# Autodesk Inventor assembly: Toughbox Nanotube 31 full gear drive
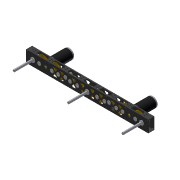
[picture p0: Inventor's stored thumbnail of the model, 180x180]
Saved by Autodesk Inventor 2013 (Build 170138000, 138)
## iProperties
Created: 2013-09-01
Part Number: Toughbox Nanotube 31 full gear drive
Document SubType Name: Assembly
Designer: Nemo
Mass: 5141.67 g
Surface Area: 5866.72 cm^2
Volume: 1617.92 cm^3
Density: 3.17795 g/cm^3
Author: Nemo
## Documents named in this file (7)
- H:\Nemo\Documents\Robotics\COTS Parts\Gearboxes\Toughbox Nanotube 31 full gear drive.iam
- H:\Nemo\Documents\Robotics\COTS Parts\Gearboxes\Components\AndyMark Housings\ToughBox Nano Tube 31.ipt
- H:\Nemo\Documents\Robotics\COTS Parts\Motors\Motor and Pinion Gear Assemblies\CIM Motor 14T.iam
- H:\Nemo\Documents\Robotics\COTS Parts\Gearboxes\50T nanotube cluster.iam
- H:\Nemo\Documents\Robotics\COTS Parts\Gearboxes\Components\50T nanotube cluster no 14T.iam
- H:\Nemo\Documents\Robotics\COTS Parts\Gearboxes\Components\24T nanotube cluster.iam
- H:\Nemo\Documents\Robotics\COTS Parts\Gearboxes\Components\Nanotube Output Cluster.iam
## Components (18 placed, 6 different names)
1. ToughBox Nano Tube 31:1 — Mate:1, Flush:1, Flush:2, Mate:3, Insert:3, Insert:6, Insert:7, Insert:8, Insert:9, Insert:10, Insert:11, Insert:12, Insert:13, Mate:4, Insert:14, Insert:15, Insert:16, Insert:17, Insert:18, Insert:19
2. CIM Motor 14T:1 [sub-assembly] — Mate:3, Insert:3
3. 50T nanotube cluster:1 [sub-assembly]
4. 50T nanotube cluster:2 [sub-assembly] — Insert:6
5. 50T nanotube cluster no 14T:1 [sub-assembly] — Insert:7
6. 50T nanotube cluster no 14T:2 [sub-assembly] — Insert:10
7. 24T nanotube cluster:1 [sub-assembly] — Insert:8
8. 24T nanotube cluster:2 [sub-assembly] — Insert:9
9. Nanotube Output Cluster:1 [sub-assembly]
10. Nanotube Output Cluster:2 [sub-assembly] — Insert:11
11. Nanotube Output Cluster:3 [sub-assembly] — Insert:12
12. CIM Motor 14T:2 [sub-assembly] — Insert:13, Mate:4
13. 50T nanotube cluster:3 [sub-assembly] — Insert:14
14. 50T nanotube cluster:4 [sub-assembly] — Insert:15
15. 50T nanotube cluster no 14T:3 [sub-assembly] — Insert:16
16. 24T nanotube cluster:3 [sub-assembly] — Insert:17
17. 24T nanotube cluster:4 [sub-assembly] — Insert:18
18. 50T nanotube cluster no 14T:4 [sub-assembly] — Insert:19
## Relationships (25: Insert 19, Mate 4, Flush 2)
- Mate:1: ToughBox Nano Tube 31:1
- Flush:1: ToughBox Nano Tube 31:1
- [Mate]: ToughBox Nano Tube 31:1 ↔ Nanotube Output Cluster:1
- [Insert]: ToughBox Nano Tube 31:1 ↔ Nanotube Output Cluster:1
- [Insert]: ToughBox Nano Tube 31:1 ↔ Nanotube Output Cluster:1
- Flush:2: ToughBox Nano Tube 31:1
- Mate:3: ToughBox Nano Tube 31:1 ↔ CIM Motor 14T:1
- Insert:3: ToughBox Nano Tube 31:1 ↔ CIM Motor 14T:1
- [Insert]: ToughBox Nano Tube 31:1 ↔ 50T nanotube cluster:1
- [Insert]: ToughBox Nano Tube 31:1 ↔ 50T nanotube cluster:1
- Insert:6: ToughBox Nano Tube 31:1 ↔ 50T nanotube cluster:2
- Insert:7: ToughBox Nano Tube 31:1 ↔ 50T nanotube cluster no 14T:1
- Insert:8: ToughBox Nano Tube 31:1 ↔ 24T nanotube cluster:1
- Insert:9: ToughBox Nano Tube 31:1 ↔ 24T nanotube cluster:2
- Insert:10: ToughBox Nano Tube 31:1 ↔ 50T nanotube cluster no 14T:2
- Insert:11: ToughBox Nano Tube 31:1 ↔ Nanotube Output Cluster:2
- Insert:12: ToughBox Nano Tube 31:1 ↔ Nanotube Output Cluster:3
- Insert:13: ToughBox Nano Tube 31:1 ↔ CIM Motor 14T:2
- Mate:4: ToughBox Nano Tube 31:1 ↔ CIM Motor 14T:2
- Insert:14: ToughBox Nano Tube 31:1 ↔ 50T nanotube cluster:3
- Insert:15: ToughBox Nano Tube 31:1 ↔ 50T nanotube cluster:4
- Insert:16: ToughBox Nano Tube 31:1 ↔ 50T nanotube cluster no 14T:3
- Insert:17: ToughBox Nano Tube 31:1 ↔ 24T nanotube cluster:3
- Insert:18: ToughBox Nano Tube 31:1 ↔ 24T nanotube cluster:4
- Insert:19: ToughBox Nano Tube 31:1 ↔ 50T nanotube cluster no 14T:4
